# Autodesk Inventor assembly: 021.5/0.25-D
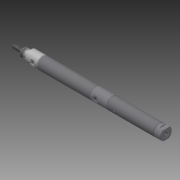
[picture p0: Inventor's stored thumbnail of the model, 180x180]
Saved by Autodesk Inventor 2014 (Build 180170000, 170)
## iProperties
Category: PARTsolutions
Company: BIMBA
Created: 2014-01-19
Part Number: 021.5/0.25-D
Catalog Web Link: www.cadenas.de
Description: Original Line Three-Position Cylinders-
Vendor: BIMBA
Document SubType Name: Assembly
Designer: Michael
Manufacturer: BIMBA
Title: 021.5/0.25-D
Author: Cadenas PARTsolutions
PSOL_IDENT_0: {$CADENAS_DATA\23d-libs\bimba\bimba\bimba_imperial\bimba_full_line\original_line_cylinders\three_pos
PSOL_IDENT_1: ition_cylinders\3position_asmtab.prj},274 {VTYP=3D},{STYP=ASSTAB},{NB=021.5/0.25-D},{LINA=021.5/0.25
PSOL_IDENT_2: -D},{NN=Original Line Three-Position Cylinders},{DATE=15.10.2013 05:44:09},{GEOMDATE=27.08.2012},{VE
PSOL_IDENT_3: RSION=},{LINEID=40},{LINESUBID=-1},{WBVAR=STROKEA,STROKEB,MNT,NR,M,NT,EE,EEL,G,K,Q,B,T,W,T1,T2,T3,T4
PSOL_IDENT_4: ,PRC,MB,MN,PB}  {NB=021.5/0.25-D},{LINA=021.5/0.25-D},{KT=DUMMY},{PN=021.5/0.25-D},{PNC=021.5/0.25-D
PSOL_IDENT_5: },{PNA=(NO ACCESSORIES)},{DASH=-},{BORE1=0.56250000},{BORE=9/16\" (02)},{BOREPN=02},{STROKEA=1.500},
PSOL_IDENT_6: {STROKEB=0.250},{STROKEALGA=[0.011:31.989/0.001]},{STROKEALGB=[0.011:30.5/0.001]},{STROKEBMAX=30.5},
PSOL_IDENT_7: {STROKE1=1.5},{STROKE2=0.250},{AC=Double Acting},{ACTING=D},{ACTINGALG= 'D' , 'Double Acting' },{ACT
PSOL_IDENT_8: INGPN=D},{MNT=},{MNTALG= '' , 'Nose Mounting (3P)' , 'XP' , 'Universal Mounting (3P)' },{MNTPN=},{TY
PSOL_IDENT_9: PE=},{NR=},{NRALG= '' , 'Round (Standard)' , 'NR' , 'Non-Rotating Square' },{NRPN=},{M=},{MALG= '', '
PSOL_IDENT_10: Without Magnet', 'M', 'With Magnet' },{MATR=303 Stainless Steel},{F=},{FALG= '', 'Non-Coated (Standa
PSOL_IDENT_11: rd)', 'F', 'Molycoated' },{FPN=},{NT=},{NTPN=},{EE=},{EEL=0.000},{EEMAX=30.250},{EEALG= '', 'Without
PSOL_IDENT_12: Extra Extension', 'EE', 'With Extra Extension' },{EELALG=0},{EEPN=},{EEPN1=0.000},{G=},{GPN=},{GPN1=
PSOL_IDENT_13: },{K=},{KALG='','N/A'},{KPN=},{Q=},{QALG= '' , 'Standard Port' , 'Q' , 'Side Port' },{QPN=},{B=},{BA
PSOL_IDENT_14: LG= '', 'Without Bumper' , 'B' , 'With Bumper' },{BPN=},{T=},{TALG= '' , 'Standard -20° to 200°F (-2
PSOL_IDENT_15: 9° to 95°C)' , 'N' , 'Low Temperature' , 'V' , 'High Temperature' },{NPN=},{VPN=},{W=},{WALG= '' , '
PSOL_IDENT_16: Without Wiper' , 'W' , 'With Wiper' },{WPN=},{E=},{EALG= '' , 'Standard Seals/Lube' , 'E' , 'Non-Lub
PSOL_IDENT_17: e Seals/Lube' },{EPN=},{ST=},{STALG= '' , 'Without Switch Track' , '-' , 'With Switch Track' },{STPA
PSOL_IDENT_18: LG= '' , 'N/A' },{STPN=},{T1=},{T2=},{T3=},{T4=},{S=},{SALG='','N/A'},{SPN=},{PRC=},{PRCALG= '' , 'w
PSOL_IDENT_19: /out Pivot Rod Clevis' , 'D-850' , 'D-850'},{PRCPN=},{MB=},{MN=},{PB=},{PBALG= '' , 'N/A' },{PBPN=},
PSOL_IDENT_20: {TLEN=3.817},{TEXT=0.2},{SPACE=0.114286},{FRAC=7.28},{BL=},{BR=},{DWGC=},{PNN=},{MNTRG=},{ACTINGRG=R
PSOL_IDENT_21: },{DIMBRL=2.28100000},{DIMBRE=1.65600000},{DIMBBL=1.00000000},{RLB=4.031},{REB=3.406},{BLB=2.750},{D
PSOL_IDENT_22: IMARL=1.85600000},{DIMARE=1.23100000},{DIMABL=0.93800000},{RLA=3.356},{REA=2.731},{BLA=2.438},{DWGCS=
PSOL_IDENT_23: D-68355},{DWGTA=D-75938},{DWGTB=D-7516},{DWGRH=D-14216},{DWGRG=D-26368},{TRANS=0.50000000},{DWGRCB=D
PSOL_IDENT_24: -7508},{DWGRCA=D-9538},{BRL=2.50000000},{BRE=1.57800000},{BBL=1.06200000},{ARL=1.91600000},{ARE=0.99
PSOL_IDENT_25: 400000},{ABL=1.06200000},{T1ALG='','N/A'},{T2ALG='','N/A'},{T3ALG='','N/A'},{T4ALG='','N/A'},{DWGST=
PSOL_IDENT_26: D-74168},{DWGS=},{STL=2.4},{TS=X},{SS=},{AA=4.12},{BA=2.25},{C=0.75},{D=#10-32},{E1=0.38},{E11=0.380
PSOL_IDENT_27: 00000},{E12=0.38000000},{F1=0.06},{G1=N/A},{H=0.50},{I=7/16-20},{J=N/A},{K1=#10-32},{L1=.434/.437},{
PSOL_IDENT_28: M1=0.19},{N=0.50},{O=0.62},{AA1=4.12000000},{BA1=2.25000000},{AA1B=4.31000000},{BA1B=2.31000000},{AA
PSOL_IDENT_29: 1XP=4.40000000},{BA1XP=2.25000000},{AA1BXP=4.59000000},{BA1BXP=2.31000000},{M11=0.19000000},{M12=0.3
PSOL_IDENT_30: 8000000},{N1=0.50000000},{N2=0.31000000},{O1=0.62000000},{O2=0.62000000},{P=N/A},{Q1=N/A},{R=N/A},{P
PSOL_IDENT_31: 1=0.25000000},{Q11=0.19000000},{R1=0.16},{MBALG= '' , 'w/out Mounting Bracket' , 'F,D-770' , 'D-770
PSOL_IDENT_32: (front)' },{MBPN=},{MBP=},{MNALG= '' , 'w/out Mounting Nut' , 'F,D-154' , 'D-154 (front)' },{MNPN=},
PSOL_IDENT_33: {MNP=},{PRCP=},{MBR=},{MBF=},{MNF=},{MNR=},{PBPNALL=},{MBPNALL=D-770},{PRCPNALL=D-850},{FNUTPN=D-154
PSOL_IDENT_34: },{RNUTPN=D-154},{ASSOPTACC=T4},{MATALGHTML=<b>Original Line Three Position:</b><dl><dt>Rod:</dt><dd
PSOL_IDENT_35: >- 303 Stainless Steel</dd><dt>Bearings:</dt><dd>- Sintered Bronze</dd><dt>Body:</dt><dd>- 304 Stain
PSOL_IDENT_36: less Steel</dd><dt>End Caps:</dt><dd>- Aluminum</dd><dt>Seals:</dt><dd>-  Buna N</dd></dl>},{PPATH=t
PSOL_IDENT_37: hree_pos_cylinder_asmtpl.prj}
CNS_NN: Original Line Three-Position Cylinders
CNS_NT: Standard Male Thread
CNS_NB: 021.5/0.25-D
CNS_NBSYN: $PNC.
CNS_LINA: 021.5/0.25-D
CNS_PN: 021.5/0.25-D
CNS_PNC: 021.5/0.25-D
CNS_PNA: (NO ACCESSORIES)
CNS_DASH: -
CNS_BORE1: 0.56250000
CNS_BORE: 9/16" [02]
CNS_BOREPN: 02
CNS_STROKEA: 1.500
CNS_STROKEB: 0.250
CNS_STROKEALGA: [0.011:31.989/0.001]
CNS_STROKEALGB: [0.011:30.5/0.001]
CNS_STROKEBMAX: 30.500
CNS_STROKE1: 1.500
CNS_STROKE2: 0.250
CNS_AC: Double
CNS_ACTING: D
CNS_ACTINGALG: 'D' , 'Double Acting'
CNS_ACTINGPN: D
CNS_MNT: Front Nose [D]
CNS_MNTALG: '' , 'Nose Mounting (3P)' , 'XP' , 'Universal Mounting (3P)'
CNS_NR: Standard Round
CNS_NRALG: '' , 'Round (Standard)' , 'NR' , 'Non-Rotating Square'
CNS_M: Without Magnet Piston
CNS_MALG: '', 'Without Magnet', 'M', 'With Magnet'
CNS_MATR: Stainless Steel
CNS_FALG: '', 'Non-Coated (Standard)', 'F', 'Molycoated'
CNS_EE: Standard Rod Extension
CNS_EEL: 0.000
CNS_EEMAX: 30.250
CNS_EEALG: '', 'Without Extra Extension', 'EE', 'With Extra Extension'
CNS_EELALG: 0
CNS_EEPN1: 0.000
CNS_G: Standard Grease Lube
CNS_K: N/A
CNS_KALG: '','N/A'
CNS_Q: Standard Axial Port
CNS_QALG: '' , 'Standard Port' , 'Q' , 'Side Port'
CNS_B: Without Bumpers
CNS_BALG: '', 'Without Bumper' , 'B' , 'With Bumper'
CNS_T: Standard -20° to 200°F (-29° to 95°C)
CNS_TALG: '' , 'Standard -20° to 200°F (-29° to 95°C)' , 'N' , 'Low Temperature' , 'V' , 'High Temperature'
CNS_W: Without Wiper
CNS_WALG: '' , 'Without Wiper' , 'W' , 'With Wiper'
CNS_EALG: '' , 'Standard Seals/Lube' , 'E' , 'Non-Lube Seals/Lube'
CNS_STALG: '' , 'Without Switch Track' , '-' , 'With Switch Track'
CNS_STPALG: '' , 'N/A'
CNS_T1: N/A
CNS_T2: N/A
CNS_T3: N/A
CNS_T4: N/A
CNS_SALG: '','N/A'
CNS_PRC: Without Piston Rod Clevis
CNS_PRCALG: '' , 'w/out Pivot Rod Clevis' , 'D-850' , 'D-850'
CNS_MB: Without Mounting Bracket
CNS_MN: Without Mounting Nut
CNS_PB: N/A
CNS_PBALG: '' , 'N/A'
CNS_TLEN: 3.817
CNS_TEXT: 0.200
CNS_SPACE: 0.114
CNS_FRAC: 7.280
CNS_ACTINGRG: R
CNS_DIMBRL: 2.28100000
CNS_DIMBRE: 1.65600000
CNS_DIMBBL: 1.00000000
CNS_RLB: 4.031
CNS_REB: 3.406
CNS_BLB: 2.750
CNS_DIMARL: 1.85600000
CNS_DIMARE: 1.23100000
CNS_DIMABL: 0.93800000
CNS_RLA: 3.356
CNS_REA: 2.731
CNS_BLA: 2.438
CNS_DWGCS: D-68355
CNS_DWGTA: D-75938
CNS_DWGTB: D-7516
CNS_DWGRH: D-14216
CNS_DWGRG: D-26368
CNS_TRANS: 0.50000000
CNS_DWGRCB: D-7508
CNS_DWGRCA: D-9538
CNS_BRL: 2.50000000
CNS_BRE: 1.57800000
CNS_BBL: 1.06200000
CNS_ARL: 1.91600000
CNS_ARE: 0.99400000
CNS_ABL: 1.06200000
CNS_T1ALG: '','N/A'
CNS_T2ALG: '','N/A'
CNS_T3ALG: '','N/A'
CNS_T4ALG: '','N/A'
CNS_DWGST: D-74168
CNS_STL: 2.400
CNS_TS: X
CNS_AA: 4.12
CNS_BA: 2.25
CNS_C: 0.75
CNS_D: #10-32
CNS_E1: 0.38
CNS_E11: 0.38000000
CNS_E12: 0.38000000
CNS_F1: 0.06
CNS_G1: N/A
CNS_H: 0.50
CNS_I: 7/16-20
CNS_J: N/A
CNS_K1: #10-32
CNS_L1: .434/.437
CNS_M1: 0.19
CNS_N: 0.50
CNS_O: 0.62
CNS_AA1: 4.12000000
CNS_BA1: 2.25000000
CNS_AA1B: 4.31000000
CNS_BA1B: 2.31000000
CNS_AA1XP: 4.40000000
CNS_BA1XP: 2.25000000
CNS_AA1BXP: 4.59000000
CNS_BA1BXP: 2.31000000
CNS_M11: 0.19000000
CNS_M12: 0.38000000
CNS_N1: 0.50000000
CNS_N2: 0.31000000
CNS_O1: 0.62000000
CNS_O2: 0.62000000
CNS_P: N/A
CNS_Q1: N/A
CNS_R: N/A
CNS_P1: 0.25000000
CNS_Q11: 0.19000000
CNS_R1: 0.16
CNS_MBALG: '' , 'w/out Mounting Bracket' , 'F,D-770' , 'D-770 (front)'
CNS_MNALG: '' , 'w/out Mounting Nut' , 'F,D-154' , 'D-154 (front)'
CNS_MBPNALL: D-770
CNS_PRCPNALL: D-850
CNS_FNUTPN: D-154
CNS_RNUTPN: D-154
CNS_ASSOPTACC: T4
CNS_MATALGHTML: <b>Original Line Three Position:</b><dl><dt>Rod:</dt><dd>- 303 Stainless Steel</dd><dt>Bearings:</dt><dd>- Sintered Bronze</dd><dt>Body:</dt><dd>- 304 Stainless Steel</dd><dt>End Caps:</dt><dd>- Aluminum</dd><dt>Seals:</dt><dd>-  Buna N</dd></dl>
CNS_PPATH: three_pos_cylinder_asmtpl.prj
SUPPLIER: BIMBA
ARTICLENO: 021.5/0.25-D
BOMINFO: 021.5/0.25-D
CREATOR: CADENAS GmbH
## Documents named in this file (9)
- C:\Users\Michael\Documents\GitHub\2014buildCAD\New Collector\021_5_0_25-D.iam
- C:\Users\Michael\Documents\GitHub\2014buildCAD\New Collector\021_5_0_25-D0_dummy.ipt
- C:\Users\Michael\Documents\GitHub\2014buildCAD\New Collector\D-68355---0.ipt
- C:\Users\Michael\Documents\GitHub\2014buildCAD\New Collector\D-75938-2_438.ipt
- C:\Users\Michael\Documents\GitHub\2014buildCAD\New Collector\D-14216rear_head.ipt
- C:\Users\Michael\Documents\GitHub\2014buildCAD\New Collector\D-7516-2_75.ipt
- C:\Users\Michael\Documents\GitHub\2014buildCAD\New Collector\D-26368----0_5_rod_guide_cyl.ipt
- C:\Users\Michael\Documents\GitHub\2014buildCAD\New Collector\D-75081_5-0_25-4_031-3pos.ipt
- C:\Users\Michael\Documents\GitHub\2014buildCAD\New Collector\D-95381_5-0_25-3_356-3pos.ipt
## Components (8 placed, 8 different names)
1. 021_5_0_25-D0_dummy:1 — dummy_XY@1 <-> centar_XY@2, dummy_Z@1 <-> centar_Z@2, dummy_YZ@1 <-> centar_YZ@2
2. D-68355---0:1 — dummy_XY@1 <-> centar_XY@2, dummy_Z@1 <-> centar_Z@2, dummy_YZ@1 <-> centar_YZ@2, to_cyl_A_XY@2 <-> tube2_XY@3, to_cyl_A_Z@2 <-> tube2_Z@3, to_cyl_A_YZ@2 <-> tube2_YZ@3, to_cyl_B_XY@2 <-> tube1_XY@5, to_cyl_B_Z@2 <-> tube1_Z@5, to_cyl_B_YZ@2 <-> tube1_YZ@5, to_rod_A_XY@2 <-> to_rod_guide_XY@8, to_rod_A_Z@2 <-> to_rod_guide_Z@8
3. D-75938-2_438:1 — to_cyl_A_XY@2 <-> tube2_XY@3, to_cyl_A_Z@2 <-> tube2_Z@3, to_cyl_A_YZ@2 <-> tube2_YZ@3, tube1_XY@3 <-> rear_head_XY@4, tube1_Z@3 <-> rear_head_Z@4, tube1_YZ@3 <-> rear_head_YZ@4
4. D-14216rear_head:1 — tube1_XY@3 <-> rear_head_XY@4, tube1_Z@3 <-> rear_head_Z@4, tube1_YZ@3 <-> rear_head_YZ@4
5. D-7516-2_75:1 — to_cyl_B_XY@2 <-> tube1_XY@5, to_cyl_B_Z@2 <-> tube1_Z@5, to_cyl_B_YZ@2 <-> tube1_YZ@5, tube2_XY@5 <-> to_tube_XY@6, tube2_Z@5 <-> to_tube_Z@6, tube2_YZ@5 <-> to_tube_YZ@6
6. D-26368----0_5_rod_guide_cyl:1 — tube2_XY@5 <-> to_tube_XY@6, tube2_Z@5 <-> to_tube_Z@6, tube2_YZ@5 <-> to_tube_YZ@6, to_rod_XY@6 <-> to_rod_guide_XY@7, to_rod_Z@6 <-> to_rod_guide_Z@7
7. D-75081_5-0_25-4_031-3pos:1 — to_rod_XY@6 <-> to_rod_guide_XY@7, to_rod_Z@6 <-> to_rod_guide_Z@7
8. D-95381_5-0_25-3_356-3pos:1 — to_rod_A_XY@2 <-> to_rod_guide_XY@8, to_rod_A_Z@2 <-> to_rod_guide_Z@8
## Relationships (19: Mate 11, Angle 5, Flush 3)
- dummy_XY@1 <-> centar_XY@2 [Mate]: 021_5_0_25-D0_dummy:1 ↔ D-68355---0:1
- dummy_Z@1 <-> centar_Z@2 [Mate]: 021_5_0_25-D0_dummy:1 ↔ D-68355---0:1
- dummy_YZ@1 <-> centar_YZ@2 [Angle] (-90 deg): 021_5_0_25-D0_dummy:1 ↔ D-68355---0:1
- to_cyl_A_XY@2 <-> tube2_XY@3 [Flush]: D-68355---0:1 ↔ D-75938-2_438:1
- to_cyl_A_Z@2 <-> tube2_Z@3 [Mate]: D-68355---0:1 ↔ D-75938-2_438:1
- to_cyl_A_YZ@2 <-> tube2_YZ@3 [Angle] (0 deg): D-68355---0:1 ↔ D-75938-2_438:1
- tube1_XY@3 <-> rear_head_XY@4 [Mate]: D-75938-2_438:1 ↔ D-14216rear_head:1
- tube1_Z@3 <-> rear_head_Z@4 [Mate]: D-75938-2_438:1 ↔ D-14216rear_head:1
- tube1_YZ@3 <-> rear_head_YZ@4 [Angle] (90 deg): D-75938-2_438:1 ↔ D-14216rear_head:1
- to_cyl_B_XY@2 <-> tube1_XY@5 [Flush]: D-68355---0:1 ↔ D-7516-2_75:1
- to_cyl_B_Z@2 <-> tube1_Z@5 [Mate]: D-68355---0:1 ↔ D-7516-2_75:1
- to_cyl_B_YZ@2 <-> tube1_YZ@5 [Angle] (0 deg): D-68355---0:1 ↔ D-7516-2_75:1
- tube2_XY@5 <-> to_tube_XY@6 [Mate]: D-7516-2_75:1 ↔ D-26368----0_5_rod_guide_cyl:1
- tube2_Z@5 <-> to_tube_Z@6 [Mate]: D-7516-2_75:1 ↔ D-26368----0_5_rod_guide_cyl:1
- tube2_YZ@5 <-> to_tube_YZ@6 [Angle] (-180 deg): D-7516-2_75:1 ↔ D-26368----0_5_rod_guide_cyl:1
- to_rod_XY@6 <-> to_rod_guide_XY@7 [Flush]: D-26368----0_5_rod_guide_cyl:1 ↔ D-75081_5-0_25-4_031-3pos:1
- to_rod_Z@6 <-> to_rod_guide_Z@7 [Mate]: D-26368----0_5_rod_guide_cyl:1 ↔ D-75081_5-0_25-4_031-3pos:1
- to_rod_A_XY@2 <-> to_rod_guide_XY@8 [Mate]: D-68355---0:1 ↔ D-95381_5-0_25-3_356-3pos:1
- to_rod_A_Z@2 <-> to_rod_guide_Z@8 [Mate]: D-68355---0:1 ↔ D-95381_5-0_25-3_356-3pos:1
